# Autodesk Inventor assembly: link0
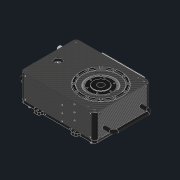
[picture p0: Inventor's stored thumbnail of the model, 180x180]
Saved by Autodesk Inventor 2022 (Build 260153000, 153)
## iProperties
Created: 2021-08-10
Part Number: link0
Document SubType Name: Assembly
Designer: yuta0
Author: yuta0
## Documents named in this file (2)
- C:\Users\yuta0\Documents\GitHub\catchrobo_hardware\mesh\link0.iam
- C:\Users\yuta0\Documents\GitHub\catchrobo_hardware\assy-robot\s-assy-link0.iam
## Components (1 placed, 1 different names)
1. s-assy-link0:1 [sub-assembly] — メイト:1, メイト:2, 角度:1
## Relationships (3: Mate 2, Angle 1)
- メイト:1 [Mate]: s-assy-link0:1
- メイト:2 [Mate]: s-assy-link0:1
- 角度:1 [Angle] (0 deg): s-assy-link0:1
